# Autodesk Inventor assembly: 775pro_3_E_1-2inHex
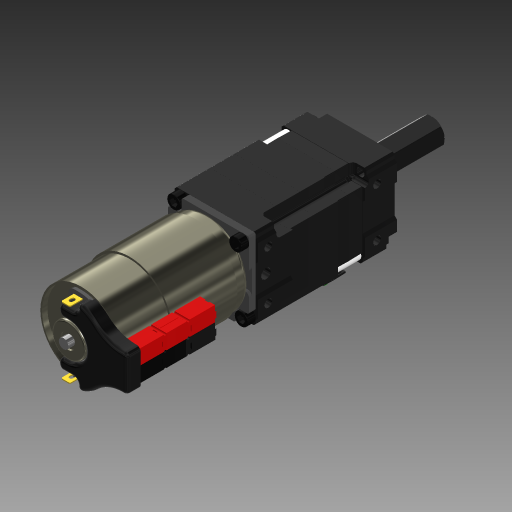
[picture p0: Inventor's stored thumbnail of the model, 512x512]
Saved by Autodesk Inventor 2023 (Build 270158000, 158)
## iProperties
Created: 2018-08-19
Part Number: 775pro_3_E_1-2inHex
Document SubType Name: Assembly
Mass: 1123.04 g
Surface Area: 1203.25 cm^2
Volume: 285.054 cm^3
Density: 3.93975 g/cm^3
## Documents named in this file (11)
- E:\Collaborative Robots\Collaborative Part Library\General Gearboxes\Planetaries\Versaplanetary\VersaPlanetary\775pro, 3 Stages, Encoder, 1-2in Hex Output.iam
- E:\Collaborative Robots\Collaborative Part Library\General Gearboxes\Planetaries\Versaplanetary\Intermediate Stages\Ring Gear.ipt
- E:\Collaborative Robots\Collaborative Part Library\General Gearboxes\Planetaries\Versaplanetary\Intermediate Stages\VP Encoder.iam
- E:\Collaborative Robots\Collaborative Part Library\General Gearboxes\Planetaries\Versaplanetary\V2 Stages\V2 Input Stage.iam
- E:\Collaborative Robots\Collaborative Part Library\General Gearboxes\Planetaries\Versaplanetary\Screws\8-32 x 2.75in Screw.ipt
- E:\Collaborative Robots\Collaborative Part Library\Power Transfer\Bearings and Bushings\Bearings\6902ZZ.ipt
- E:\Middleton Robotics\Collaborative Robots\Colaborative Part Library\General Gearboxes\Planetaries\Versaplanetary\V2 Stages\V2 Output Stage.iam
- E:\Middleton Robotics\Collaborative Robots\Collaborative Part Library\Power Transfer\Bearings.ipt
- E:\Collaborative Robots\Collaborative Part Library\General Gearboxes\Planetaries\Versaplanetary\V2 Stages\V2 Output Stage\VP V2 Output Stage 1-2in Hex.iam
- E:\Collaborative Robots\Collaborative Part Library\General Gearboxes\Planetaries\Versaplanetary\V2 Stages\V2 Input Stage\VP 775pro Input.iam
- E:\Collaborative Robots\Collaborative Part Library\General Gearboxes\Planetaries\Versaplanetary\VersaPlanetary.iam
## Components (9 placed, 7 different names)
1. VP V2 Output Stage 1-2in Hex:1 [sub-assembly] — EncoderConstraint1, EncoderConstraint2, EncoderConstraint3, Flush:6, 3StageBasicInputMate2, Insert:25
2. Ring Gear 2 — Insert:3, Flush:2, Mate:4, Mate:5, Flush:6
3. Ring Gear 3 — Insert:3, Flush:2, 3StageBasicInputMate1
4. VP Encoder:1 [sub-assembly] — EncoderConstraint1, EncoderConstraint2, EncoderConstraint3, Mate:4, Mate:5
5. VP 775pro Input:1 [sub-assembly] — 3StageBasicInputMate1, 3StageBasicInputMate2, Insert:14, Insert:15
6. 8-32 x 2.75in Screw:1 — Insert:14
7. 8-32 x 2.75in Screw:2 — Insert:15
8. 6902ZZ:1
9. 6902ZZ:2 — Insert:25
## Relationships (13: Insert 5, Mate 4, Flush 3, Angle 1)
- Insert:3: Ring Gear 2 ↔ Ring Gear 3
- Flush:2: Ring Gear 2 ↔ Ring Gear 3
- EncoderConstraint1 [Mate]: VP V2 Output Stage 1-2in Hex:1 ↔ VP Encoder:1
- EncoderConstraint2 [Mate]: VP V2 Output Stage 1-2in Hex:1 ↔ VP Encoder:1
- EncoderConstraint3 [Angle] (0 deg): VP V2 Output Stage 1-2in Hex:1 ↔ VP Encoder:1
- Mate:4: Ring Gear 2 ↔ VP Encoder:1
- Mate:5: Ring Gear 2 ↔ VP Encoder:1
- Flush:6: VP V2 Output Stage 1-2in Hex:1 ↔ Ring Gear 2
- 3StageBasicInputMate1 [Insert]: Ring Gear 3 ↔ VP 775pro Input:1
- 3StageBasicInputMate2 [Flush]: VP V2 Output Stage 1-2in Hex:1 ↔ VP 775pro Input:1
- Insert:14: VP 775pro Input:1 ↔ 8-32 x 2.75in Screw:1
- Insert:15: VP 775pro Input:1 ↔ 8-32 x 2.75in Screw:2
- Insert:25: VP V2 Output Stage 1-2in Hex:1 ↔ 6902ZZ:2
